# Autodesk Inventor assembly: practice
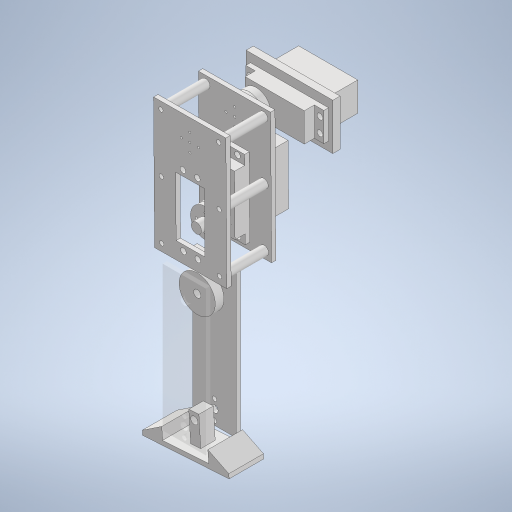
[picture p0: Inventor's stored thumbnail of the model, 512x512]
Saved by Autodesk Inventor 2024.3 (Build 283343000, 343)
## iProperties
Created: 2024-10-22
Part Number: practice
Document SubType Name: Assembly
Designer: 佐藤智貴
Author: 佐藤智貴
## Documents named in this file (11)
- C:\Users\佐藤智貴\OneDrive - Chiba Institute of Technology\ドキュメント\Inventor\Biped_robot\practice.iam
- C:\Users\佐藤智貴\OneDrive - Chiba Institute of Technology\ドキュメント\Inventor\Biped_robot\servo.ipt
- C:\Users\佐藤智貴\OneDrive - Chiba Institute of Technology\ドキュメント\Inventor\Biped_robot\gear_01.ipt
- C:\Users\佐藤智貴\OneDrive - Chiba Institute of Technology\ドキュメント\Inventor\Biped_robot\servo_case.ipt
- C:\Users\佐藤智貴\OneDrive - Chiba Institute of Technology\ドキュメント\Inventor\Biped_robot\practice_parts01.ipt
- C:\Users\佐藤智貴\OneDrive - Chiba Institute of Technology\ドキュメント\Inventor\Biped_robot\practice_parts02.ipt
- C:\Users\佐藤智貴\OneDrive - Chiba Institute of Technology\ドキュメント\Inventor\Biped_robot\servo_horn.ipt
- C:\Users\佐藤智貴\OneDrive - Chiba Institute of Technology\ドキュメント\Inventor\Biped_robot\spacer_28mm.ipt
- C:\Users\佐藤智貴\OneDrive - Chiba Institute of Technology\ドキュメント\Inventor\Biped_robot\gear_02.ipt
- C:\Users\佐藤智貴\OneDrive - Chiba Institute of Technology\ドキュメント\Inventor\Biped_robot\practice_parts03.ipt
- C:\Users\佐藤智貴\OneDrive - Chiba Institute of Technology\ドキュメント\Inventor\Biped_robot\sole_practice.ipt
## Components (18 placed, 10 different names)
1. servo:1 — 挿入:1, 挿入:2, 挿入:3
2. servo_case:1 — 挿入:1, 挿入:2
3. servo_horn:1 — 挿入:3, 挿入:22, 挿入:23
4. practice_parts01:1 — 挿入:6, 挿入:7, 挿入:11, 挿入:12, 挿入:13, 挿入:14, 挿入:19, 挿入:20, 挿入:21, 挿入:24, 挿入:25
5. servo:2 — 挿入:6, 挿入:7, 挿入:8
6. servo_horn:2 — 挿入:8, 挿入:9, 挿入:10
7. gear_01:1 — 挿入:9, 挿入:10
8. practice_parts01:2 — 挿入:11, 挿入:12
9. spacer_28mm:1 — 挿入:20
10. spacer_28mm:2 — 挿入:14
11. spacer_28mm:3 — 挿入:13
12. spacer_28mm:4 — 挿入:19
13. gear_02:1 — 挿入:17, 挿入:18
14. practice_parts02:1 — 挿入:18, 挿入:26
15. practice_parts02:2 — 挿入:17, 挿入:27
16. spacer_28mm:5 — 挿入:21
17. practice_parts03:1 — 挿入:22, 挿入:23, 挿入:24, 挿入:25
18. sole_practice:1 — 挿入:26, 挿入:27
## Relationships (23: Insert 23)
- 挿入:1 [Insert]: servo:1 ↔ servo_case:1
- 挿入:2 [Insert]: servo:1 ↔ servo_case:1
- 挿入:3 [Insert]: servo:1 ↔ servo_horn:1
- 挿入:6 [Insert]: practice_parts01:1 ↔ servo:2
- 挿入:7 [Insert]: practice_parts01:1 ↔ servo:2
- 挿入:8 [Insert]: servo:2 ↔ servo_horn:2
- 挿入:9 [Insert]: servo_horn:2 ↔ gear_01:1
- 挿入:10 [Insert]: servo_horn:2 ↔ gear_01:1
- 挿入:11 [Insert] (28 mm): practice_parts01:1 ↔ practice_parts01:2
- 挿入:12 [Insert] (28 mm): practice_parts01:1 ↔ practice_parts01:2
- 挿入:13 [Insert]: practice_parts01:1 ↔ spacer_28mm:3
- 挿入:14 [Insert]: practice_parts01:1 ↔ spacer_28mm:2
- 挿入:17 [Insert] (6 mm): gear_02:1 ↔ practice_parts02:2
- 挿入:18 [Insert] (6 mm): gear_02:1 ↔ practice_parts02:1
- 挿入:19 [Insert]: practice_parts01:1 ↔ spacer_28mm:4
- 挿入:20 [Insert]: practice_parts01:1 ↔ spacer_28mm:1
- 挿入:21 [Insert]: practice_parts01:1 ↔ spacer_28mm:5
- 挿入:22 [Insert]: servo_horn:1 ↔ practice_parts03:1
- 挿入:23 [Insert]: servo_horn:1 ↔ practice_parts03:1
- 挿入:24 [Insert]: practice_parts01:1 ↔ practice_parts03:1
- 挿入:25 [Insert]: practice_parts01:1 ↔ practice_parts03:1
- 挿入:26 [Insert] (4 mm): practice_parts02:1 ↔ sole_practice:1
- 挿入:27 [Insert] (4 mm): practice_parts02:2 ↔ sole_practice:1
